# Autodesk Inventor assembly: Assembly Sensor Module
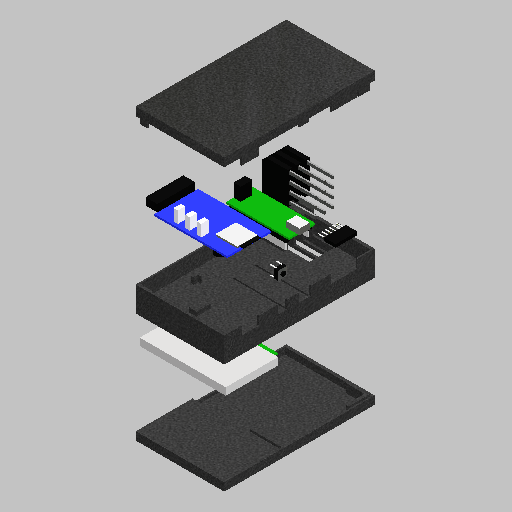
[picture p0: Inventor's stored thumbnail of the model, 512x512]
Saved by Autodesk Inventor 2025.2 (Build 292293000, 293)
## iProperties
Created: 2025-04-04
Part Number: Assembly Sensor Module
Document SubType Name: Assembly
Designer: joaki
Mass: 70.9221 g
Surface Area: 774.353 cm^2
Volume: 70.9221 cm^3
Density: 1 g/cm^3
Author: joaki
## Documents named in this file (12)
- C:\Users\joaki\OneDrive\Dokumenter\Inventor\namo\ASSEMBLED SENSOR MODULE.iam
- C:\Users\joaki\OneDrive\Dokumenter\Inventor\namo\middle plate.ipt
- C:\Users\joaki\OneDrive\Dokumenter\Inventor\namo\nano.ipt
- C:\Users\joaki\OneDrive\Dokumenter\Inventor\namo\Sd card reader.ipt
- C:\Users\joaki\OneDrive\Dokumenter\Inventor\namo\button.ipt
- C:\Users\joaki\OneDrive\Dokumenter\Inventor\namo\Rectifier.ipt
- C:\Users\joaki\OneDrive\Dokumenter\Inventor\namo\connector.ipt
- C:\Users\joaki\OneDrive\Dokumenter\Inventor\namo\Battery.ipt
- C:\Users\joaki\OneDrive\Dokumenter\Inventor\namo\battery connector.ipt
- C:\Users\joaki\OneDrive\Dokumenter\Inventor\namo\Boost converter.ipt
- C:\Users\joaki\OneDrive\Dokumenter\Inventor\namo\lid top.ipt
- C:\Users\joaki\OneDrive\Dokumenter\Inventor\namo\Lid bottom.ipt
## Components (13 placed, 11 different names)
1. middle plate:1 — Rigid:1, Rigid:3, Rigid:10, Rigid:11, Rigid:12, Rigid:13, Rigid:14, Rigid:15, Rigid:16, Rigid:17, Rigid:18, Rigid:19
2. nano:1 — Rigid:1
3. Sd card reader:1 — Rigid:16
4. button:1 — Rigid:3
5. Rectifier:1 — Rigid:19
6. Rectifier:2 — Rigid:18
7. Rectifier:3 — Rigid:17
8. connector:1 — Rigid:15
9. Battery:1 — Rigid:14
10. battery connector:1 — Rigid:10
11. Boost converter:1 — Rigid:11
12. lid top:1 — Rigid:12
13. Lid bottom:1 — Rigid:13
## Relationships (12: WeldJoint 12)
- Rigid:1 [WeldJoint] (40 mm): middle plate:1 ↔ nano:1
- Rigid:3 [WeldJoint] (20 mm): middle plate:1 ↔ button:1
- Rigid:10 [WeldJoint] (40 mm): middle plate:1 ↔ battery connector:1
- Rigid:11 [WeldJoint] (60 mm): middle plate:1 ↔ Boost converter:1
- Rigid:12 [WeldJoint] (100 mm): middle plate:1 ↔ lid top:1
- Rigid:13 [WeldJoint] (70 mm): middle plate:1 ↔ Lid bottom:1
- Rigid:14 [WeldJoint] (20 mm): middle plate:1 ↔ Battery:1
- Rigid:15 [WeldJoint] (20 mm): middle plate:1 ↔ connector:1
- Rigid:16 [WeldJoint] (50 mm): middle plate:1 ↔ Sd card reader:1
- Rigid:17 [WeldJoint] (10 mm): middle plate:1 ↔ Rectifier:3
- Rigid:18 [WeldJoint] (10 mm): middle plate:1 ↔ Rectifier:2
- Rigid:19 [WeldJoint] (10 mm): middle plate:1 ↔ Rectifier:1
